# Autodesk Inventor assembly: shooter_MIR
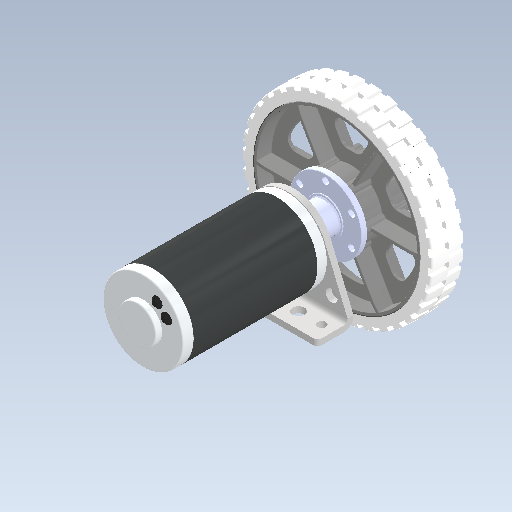
[picture p0: Inventor's stored thumbnail of the model, 512x512]
Saved by Autodesk Inventor 2020.2 (Build 242310000, 310)
## iProperties
Created: 2020-01-12
Part Number: shooter_MIR
Document SubType Name: Assembly
Designer: robst
Author: robst
## Documents named in this file (5)
- C:\git\CAD-Development\robSteele\2020LongRobotBase\shooter_MIR.iam
- C:\git\CAD-Development\robSteele\2020LongRobotBase\am-0255 2.5inch CIM Motor_MIR.ipt
- C:\git\CAD-Development\robSteele\2020LongRobotBase\6 HiGrip Asm Rev II_MIR.iam
- C:\git\CAD-Development\robSteele\2020LongRobotBase\AM 2488 CIM bracket_MIR.ipt
- C:\git\CAD-Development\robSteele\2020LongRobotBase\am-0320a_8mm_Key_Hub_MIR.ipt
## Components (4 placed, 4 different names)
1. am-0255 2.5inch CIM Motor_MIR:1 — Insert:2, Insert:1, Insert:3
2. 6 HiGrip Asm Rev II_MIR:1 [sub-assembly] — Insert:4, Mate:1
3. AM 2488 CIM bracket_MIR:1 — Insert:2, Insert:1, Angle:1
4. am-0320a_8mm_Key_Hub_MIR:1 — Insert:4, Insert:3
## Relationships (6: Insert 4, Angle 1, Mate 1)
- Insert:2: am-0255 2.5inch CIM Motor_MIR:1 ↔ AM 2488 CIM bracket_MIR:1
- Insert:1: am-0255 2.5inch CIM Motor_MIR:1 ↔ AM 2488 CIM bracket_MIR:1
- Insert:4: 6 HiGrip Asm Rev II_MIR:1 ↔ am-0320a_8mm_Key_Hub_MIR:1
- Insert:3: am-0255 2.5inch CIM Motor_MIR:1 ↔ am-0320a_8mm_Key_Hub_MIR:1
- Angle:1 (0 deg): AM 2488 CIM bracket_MIR:1
- Mate:1: 6 HiGrip Asm Rev II_MIR:1
